# Autodesk Inventor assembly: Frame_350x350
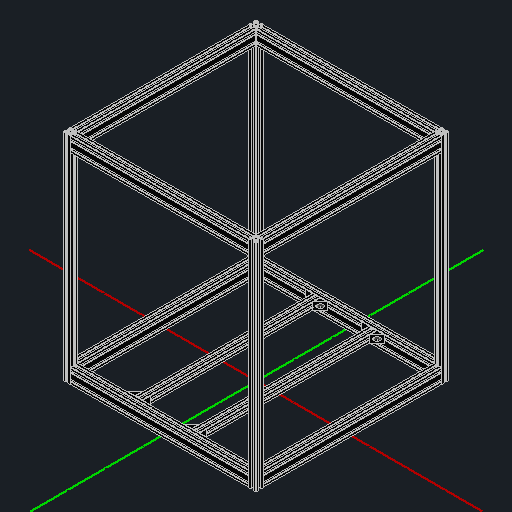
[picture p0: Inventor's stored thumbnail of the model, 512x512]
Saved by Autodesk Inventor 2022 (Build 260153000, 153)
## iProperties
Created: 2022-03-06
Part Number: Frame_350x350
Document SubType Name: Assembly
Designer: sleib
Author: sleib
## Documents named in this file (5)
- C:\Users\sleib\Projekte\Voron-2\CAD\Inventor\Frame 350x350.iam
- C:\Users\sleib\Projekte\Voron-2\CAD\Inventor\Extrusion 20x40x470.ipt
- C:\Users\sleib\Projekte\Voron-2\CAD\Inventor\Extrusion 20x20x570.ipt
- C:\Users\sleib\Projekte\Voron-2\CAD\Inventor\Extrusion 20x20x470.ipt
- C:\Users\sleib\Projekte\Voron-2\CAD\Inventor\90deg Corner (OpenBuilds).iam
## Components (22 placed, 4 different names)
1. Extrusion 20x40x470:1 — Passend:1, Fluchtend:1, Fluchtend:2, Passend:3, Fluchtend:5, Fluchtend:6, Symmetrie:2, Passend:13, Passend:14, Fluchtend:23, Fluchtend:24, Passend:15, Passend:17, Passend:19, Passend:21
2. Extrusion 20x40x470:2 — Passend:2, Fluchtend:3, Fluchtend:4
3. Extrusion 20x40x470:3 — Passend:4, Fluchtend:7, Fluchtend:8, Symmetrie:2, Passend:23, Passend:24, Passend:27, Passend:28
4. Extrusion 20x40x470:4 — Passend:5, Fluchtend:9, Fluchtend:10, Fluchtend:11, Fluchtend:12, Passend:6
5. Extrusion 20x20x570:1 — Passend:1, Fluchtend:1, Fluchtend:2, Passend:2, Fluchtend:3, Fluchtend:4, Passend:7, Fluchtend:13, Fluchtend:14, Passend:11, Fluchtend:21, Fluchtend:22, Passend:12
6. Extrusion 20x20x570:2 — Passend:3, Fluchtend:5, Fluchtend:6, Passend:9, Fluchtend:17, Fluchtend:18, Passend:10, Fluchtend:19, Fluchtend:20
7. Extrusion 20x20x570:3 — Passend:4, Fluchtend:7, Fluchtend:8, Passend:5, Fluchtend:9, Fluchtend:10, Fluchtend:15, Fluchtend:16, Passend:8
8. Extrusion 20x20x570:4 — Fluchtend:11, Fluchtend:12, Passend:6
9. Extrusion 20x40x470:5 — Passend:7, Fluchtend:13, Fluchtend:14, Fluchtend:15, Fluchtend:16, Passend:8, Symmetrie:1
10. Extrusion 20x40x470:6 — Passend:10, Fluchtend:19, Fluchtend:20
11. Extrusion 20x40x470:7 — Passend:9, Fluchtend:17, Fluchtend:18, Symmetrie:1
12. Extrusion 20x40x470:8 — Passend:11, Fluchtend:21, Fluchtend:22
13. Extrusion 20x20x470:1 — Passend:13, Fluchtend:24, Symmetrie:3, Fluchtend:25, Passend:16, Fluchtend:26, Fluchtend:27, Passend:18, Passend:29, Passend:30, Fluchtend:30, Fluchtend:31
14. Extrusion 20x20x470:2 — Passend:14, Fluchtend:23, Symmetrie:3, Fluchtend:25, Passend:20, Passend:22, Fluchtend:28, Fluchtend:29, Passend:25, Passend:26, Fluchtend:32, Fluchtend:33
15. 90deg Corner (OpenBuilds):1 [sub-assembly] — Passend:19, Passend:20, Fluchtend:29
16. 90deg Corner (OpenBuilds):2 [sub-assembly] — Passend:21, Passend:22, Fluchtend:28
17. 90deg Corner (OpenBuilds):3 [sub-assembly] — Fluchtend:27, Passend:17, Passend:18
18. 90deg Corner (OpenBuilds):4 [sub-assembly] — Passend:15, Passend:16, Fluchtend:26
19. 90deg Corner (OpenBuilds):5 [sub-assembly] — Passend:28, Passend:29, Fluchtend:30
20. 90deg Corner (OpenBuilds):6 [sub-assembly] — Passend:27, Passend:30, Fluchtend:31
21. 90deg Corner (OpenBuilds):7 [sub-assembly] — Passend:24, Passend:25, Fluchtend:32
22. 90deg Corner (OpenBuilds):8 [sub-assembly] — Passend:23, Passend:26, Fluchtend:33
## Relationships (66: Flush 33, Mate 30, Symmetry 3)
- Passend:1 [Mate]: Extrusion 20x40x470:1 ↔ Extrusion 20x20x570:1
- Fluchtend:1 [Flush]: Extrusion 20x40x470:1 ↔ Extrusion 20x20x570:1
- Fluchtend:2 [Flush]: Extrusion 20x40x470:1 ↔ Extrusion 20x20x570:1
- Passend:2 [Mate]: Extrusion 20x40x470:2 ↔ Extrusion 20x20x570:1
- Fluchtend:3 [Flush]: Extrusion 20x40x470:2 ↔ Extrusion 20x20x570:1
- Fluchtend:4 [Flush]: Extrusion 20x40x470:2 ↔ Extrusion 20x20x570:1
- Passend:3 [Mate]: Extrusion 20x40x470:1 ↔ Extrusion 20x20x570:2
- Fluchtend:5 [Flush]: Extrusion 20x40x470:1 ↔ Extrusion 20x20x570:2
- Fluchtend:6 [Flush]: Extrusion 20x40x470:1 ↔ Extrusion 20x20x570:2
- Passend:4 [Mate]: Extrusion 20x40x470:3 ↔ Extrusion 20x20x570:3
- Fluchtend:7 [Flush]: Extrusion 20x40x470:3 ↔ Extrusion 20x20x570:3
- Fluchtend:8 [Flush]: Extrusion 20x40x470:3 ↔ Extrusion 20x20x570:3
- Passend:5 [Mate]: Extrusion 20x40x470:4 ↔ Extrusion 20x20x570:3
- Fluchtend:9 [Flush]: Extrusion 20x40x470:4 ↔ Extrusion 20x20x570:3
- Fluchtend:10 [Flush]: Extrusion 20x40x470:4 ↔ Extrusion 20x20x570:3
- Fluchtend:11 [Flush]: Extrusion 20x40x470:4 ↔ Extrusion 20x20x570:4
- Fluchtend:12 [Flush]: Extrusion 20x40x470:4 ↔ Extrusion 20x20x570:4
- Passend:6 [Mate]: Extrusion 20x40x470:4 ↔ Extrusion 20x20x570:4
- Passend:7 [Mate]: Extrusion 20x20x570:1 ↔ Extrusion 20x40x470:5
- Fluchtend:13 [Flush]: Extrusion 20x20x570:1 ↔ Extrusion 20x40x470:5
- Fluchtend:14 [Flush]: Extrusion 20x20x570:1 ↔ Extrusion 20x40x470:5
- Fluchtend:15 [Flush]: Extrusion 20x20x570:3 ↔ Extrusion 20x40x470:5
- Fluchtend:16 [Flush]: Extrusion 20x20x570:3 ↔ Extrusion 20x40x470:5
- Passend:8 [Mate]: Extrusion 20x20x570:3 ↔ Extrusion 20x40x470:5
- Passend:9 [Mate]: Extrusion 20x20x570:2 ↔ Extrusion 20x40x470:7
- Fluchtend:17 [Flush]: Extrusion 20x20x570:2 ↔ Extrusion 20x40x470:7
- Fluchtend:18 [Flush]: Extrusion 20x20x570:2 ↔ Extrusion 20x40x470:7
- Passend:10 [Mate]: Extrusion 20x20x570:2 ↔ Extrusion 20x40x470:6
- Fluchtend:19 [Flush]: Extrusion 20x20x570:2 ↔ Extrusion 20x40x470:6
- Fluchtend:20 [Flush]: Extrusion 20x20x570:2 ↔ Extrusion 20x40x470:6
- Passend:11 [Mate]: Extrusion 20x20x570:1 ↔ Extrusion 20x40x470:8
- Fluchtend:21 [Flush]: Extrusion 20x20x570:1 ↔ Extrusion 20x40x470:8
- Fluchtend:22 [Flush]: Extrusion 20x20x570:1 ↔ Extrusion 20x40x470:8
- Passend:12 [Mate]: Extrusion 20x20x570:1
- Symmetrie:1: Extrusion 20x40x470:5 ↔ Extrusion 20x40x470:7
- Symmetrie:2: Extrusion 20x40x470:1 ↔ Extrusion 20x40x470:3
- Passend:13 [Mate]: Extrusion 20x40x470:1 ↔ Extrusion 20x20x470:1
- Passend:14 [Mate]: Extrusion 20x40x470:1 ↔ Extrusion 20x20x470:2
- Fluchtend:23 [Flush]: Extrusion 20x40x470:1 ↔ Extrusion 20x20x470:2
- Fluchtend:24 [Flush]: Extrusion 20x40x470:1 ↔ Extrusion 20x20x470:1
- Symmetrie:3: Extrusion 20x20x470:1 ↔ Extrusion 20x20x470:2
- Fluchtend:25 [Flush] (150 mm): Extrusion 20x20x470:1 ↔ Extrusion 20x20x470:2
- Passend:15 [Mate]: Extrusion 20x40x470:1 ↔ 90deg Corner (OpenBuilds):4
- Passend:16 [Mate]: Extrusion 20x20x470:1 ↔ 90deg Corner (OpenBuilds):4
- Fluchtend:26 [Flush]: Extrusion 20x20x470:1 ↔ 90deg Corner (OpenBuilds):4
- Fluchtend:27 [Flush]: Extrusion 20x20x470:1 ↔ 90deg Corner (OpenBuilds):3
- Passend:17 [Mate]: Extrusion 20x40x470:1 ↔ 90deg Corner (OpenBuilds):3
- Passend:18 [Mate]: Extrusion 20x20x470:1 ↔ 90deg Corner (OpenBuilds):3
- Passend:19 [Mate]: Extrusion 20x40x470:1 ↔ 90deg Corner (OpenBuilds):1
- Passend:20 [Mate]: Extrusion 20x20x470:2 ↔ 90deg Corner (OpenBuilds):1
- Passend:21 [Mate]: Extrusion 20x40x470:1 ↔ 90deg Corner (OpenBuilds):2
- Passend:22 [Mate]: Extrusion 20x20x470:2 ↔ 90deg Corner (OpenBuilds):2
- Fluchtend:28 [Flush]: Extrusion 20x20x470:2 ↔ 90deg Corner (OpenBuilds):2
- Fluchtend:29 [Flush]: Extrusion 20x20x470:2 ↔ 90deg Corner (OpenBuilds):1
- Passend:23 [Mate]: Extrusion 20x40x470:3 ↔ 90deg Corner (OpenBuilds):8
- Passend:24 [Mate]: Extrusion 20x40x470:3 ↔ 90deg Corner (OpenBuilds):7
- Passend:25 [Mate]: Extrusion 20x20x470:2 ↔ 90deg Corner (OpenBuilds):7
- Passend:26 [Mate]: Extrusion 20x20x470:2 ↔ 90deg Corner (OpenBuilds):8
- Passend:27 [Mate]: Extrusion 20x40x470:3 ↔ 90deg Corner (OpenBuilds):6
- Passend:28 [Mate]: Extrusion 20x40x470:3 ↔ 90deg Corner (OpenBuilds):5
- Passend:29 [Mate]: Extrusion 20x20x470:1 ↔ 90deg Corner (OpenBuilds):5
- Passend:30 [Mate]: Extrusion 20x20x470:1 ↔ 90deg Corner (OpenBuilds):6
- Fluchtend:30 [Flush]: Extrusion 20x20x470:1 ↔ 90deg Corner (OpenBuilds):5
- Fluchtend:31 [Flush]: Extrusion 20x20x470:1 ↔ 90deg Corner (OpenBuilds):6
- Fluchtend:32 [Flush]: Extrusion 20x20x470:2 ↔ 90deg Corner (OpenBuilds):7
- Fluchtend:33 [Flush]: Extrusion 20x20x470:2 ↔ 90deg Corner (OpenBuilds):8
